# Autodesk Inventor assembly: Arm Rod
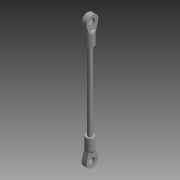
[picture p0: Inventor's stored thumbnail of the model, 180x180]
Saved by Autodesk Inventor 2014 SP1 (Build 180222100, 222)
## iProperties
Created: 2013-12-29
Part Number: Arm Rod
Document SubType Name: Assembly
Designer: tom
Author: tom
## Documents named in this file (3)
- C:\Users\tom\Documents\GitHub\Delta_Robots\Delatabot - Small Model\Inventor\Deltabot - Small Model\Arm Rod.iam
- C:\Users\tom\Documents\GitHub\Delta_Robots\Delatabot - Small Model\Inventor\Deltabot - Small Model\Body.ipt
- C:\Users\tom\Documents\rod.ipt
## Components (3 placed, 2 different names)
1. Body:1 — Flush:1
2. Body:2
3. rod:1 — Flush:1
## Relationships (1: Flush 1)
- Flush:1: Body:1 ↔ rod:1
